# Autodesk Inventor assembly: Adrian_Rolle
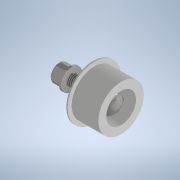
[picture p0: Inventor's stored thumbnail of the model, 180x180]
Saved by Autodesk Inventor 2021 (Build 250183000, 183)
## iProperties
Created: 2022-07-12
Part Number: Adrian_Rolle
Document SubType Name: Assembly
Designer: adria
Mass: 54.4715 g
Surface Area: 105.792 cm^2
Volume: 16.791 cm^3
Density: 3.24409 g/cm^3
Author: adria
## Documents named in this file (6)
- C:\Users\adria\OneDrive - tum.de\G2_Waste-Recycling\CAD\Adrian_Rolle.iam
- C:\Users\adria\OneDrive - tum.de\G2_Waste-Recycling\CAD\SKF_608.iam
- C:\Users\adria\OneDrive - tum.de\G2_Waste-Recycling\CAD\Rolle_schieber22.2.ipt
- C:\Users\adria\Documents\Inventor\Content Center Files\R2021\de-DE\ISO 4034(2)\ISO 4034 - M8 - ISO.ipt
- C:\Users\adria\Documents\Inventor\Content Center Files\R2021\de-DE\DIN 125-1  A\DIN 125 - A 8,4.ipt
- C:\Users\adria\Documents\Inventor\Content Center Files\R2021\de-DE\ANSI B18.3.1M(6)\ANSI B18.3.1M - M8x1,25 x 35(1).ipt
## Components (6 placed, 5 different names)
1. SKF_608:1 [sub-assembly] — Passend:1, Passend:5, Passend:6, Fluchtend:1
2. Rolle_schieber22.2:1 — Passend:1, Passend:8, Fluchtend:1, Passend:9
3. ISO 4034 M8:1 — Passend:7
4. DIN 125-1 A A 8,4:1 — Passend:8, Passend:10
5. DIN 125-1 A A 8,4:2 — Passend:5, Passend:6, Passend:7
6. Zylinderschraube mit geschmiedetem Innensechskant - Metrisch M8x1,25 x 35:1 — Passend:9, Passend:10
## Relationships (8: Mate 7, Flush 1)
- Passend:1 [Mate]: SKF_608:1 ↔ Rolle_schieber22.2:1
- Passend:5 [Mate]: SKF_608:1 ↔ DIN 125-1 A A 8,4:2
- Passend:6 [Mate]: SKF_608:1 ↔ DIN 125-1 A A 8,4:2
- Passend:7 [Mate]: ISO 4034 M8:1 ↔ DIN 125-1 A A 8,4:2
- Passend:8 [Mate] (16 mm): Rolle_schieber22.2:1 ↔ DIN 125-1 A A 8,4:1
- Fluchtend:1 [Flush]: SKF_608:1 ↔ Rolle_schieber22.2:1
- Passend:9 [Mate]: Rolle_schieber22.2:1 ↔ Zylinderschraube mit geschmiedetem Innensechskant - Metrisch M8x1,25 x 35:1
- Passend:10 [Mate]: DIN 125-1 A A 8,4:1 ↔ Zylinderschraube mit geschmiedetem Innensechskant - Metrisch M8x1,25 x 35:1
